# Autodesk Inventor assembly: Spark Max and Bracket
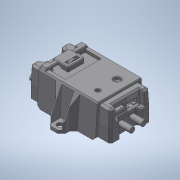
[picture p0: Inventor's stored thumbnail of the model, 180x180]
Saved by Autodesk Inventor 2022.3 (Build 263350000, 350)
## iProperties
Created: 2023-02-11
Part Number: Spark Max and Bracket
Document SubType Name: Assembly
Designer: mavericks
Author: mavericks
## Documents named in this file (3)
- T:\EIT\2023 Charged Up\COMMON PARTS\ELECTRONICS\Rev Robotics\Spark Max and Bracket.iam
- T:\EIT\2023 Charged Up\COMMON PARTS\ELECTRONICS\Rev Robotics\Spark MaxREV-11-2158.ipt
- T:\EIT\2023 Charged Up\COMMON PARTS\ELECTRONICS\Rev Robotics\SPARK_MAX_BRACKETREV-21-2151.ipt
## Components (2 placed, 2 different names)
1. SPARK_MAX_BRACKETREV-21-2151:1 — Mate:1, Mate:2, Flush:1
2. Spark MaxREV-11-2158:1 — Mate:1, Mate:2, Flush:1
## Relationships (3: Mate 2, Flush 1)
- Mate:1: SPARK_MAX_BRACKETREV-21-2151:1 ↔ Spark MaxREV-11-2158:1
- Mate:2: SPARK_MAX_BRACKETREV-21-2151:1 ↔ Spark MaxREV-11-2158:1
- Flush:1: SPARK_MAX_BRACKETREV-21-2151:1 ↔ Spark MaxREV-11-2158:1
